# Autodesk Inventor assembly: GripperAssy
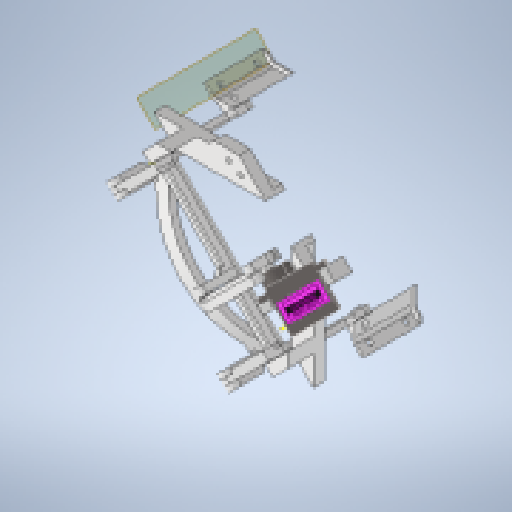
[picture p0: Inventor's stored thumbnail of the model, 512x512]
Saved by Autodesk Inventor 2025.1 (Build 291241000, 241)
## iProperties
Created: 2026-05-06
Part Number: GripperAssy
Document SubType Name: Assembly
Designer: User
Author: User
## Documents named in this file (13)
- D:\One Drive\OneDrive - Politeknik Sultan Salahuddin Abdul Aziz Shah\Documents\Inventor\RobosotPSA\GripperAssy.iam
- D:\One Drive\OneDrive - Politeknik Sultan Salahuddin Abdul Aziz Shah\Documents\Inventor\RobosotPSA\Dribbler_v2.ipt
- D:\One Drive\OneDrive - Politeknik Sultan Salahuddin Abdul Aziz Shah\Documents\Inventor\RobosotPSA\M90S_ali\M90S_ali\M90S_ali.ipt
- D:\One Drive\OneDrive - Politeknik Sultan Salahuddin Abdul Aziz Shah\Documents\Inventor\RobosotPSA\MG90S_arm01\MG90S_arm01\MG90S_arm01.ipt
- D:\One Drive\OneDrive - Politeknik Sultan Salahuddin Abdul Aziz Shah\Documents\Inventor\RobosotPSA\Gripper.ipt
- D:\One Drive\OneDrive - Politeknik Sultan Salahuddin Abdul Aziz Shah\Documents\Inventor\RobosotPSA\ServoShaft.ipt
- D:\One Drive\OneDrive - Politeknik Sultan Salahuddin Abdul Aziz Shah\Documents\Inventor\RobosotPSA\GripperHandleRight.ipt
- D:\One Drive\OneDrive - Politeknik Sultan Salahuddin Abdul Aziz Shah\Documents\Inventor\RobosotPSA\GripperHandleLeft.ipt
- D:\One Drive\OneDrive - Politeknik Sultan Salahuddin Abdul Aziz Shah\Documents\Inventor\RobosotPSA\Gripper_v1.ipt
- D:\One Drive\OneDrive - Politeknik Sultan Salahuddin Abdul Aziz Shah\Documents\Inventor\RobosotPSA\GripperShaftRight.ipt
- D:\One Drive\OneDrive - Politeknik Sultan Salahuddin Abdul Aziz Shah\Documents\Inventor\RobosotPSA\GripperShaftLeft.ipt
- D:\One Drive\OneDrive - Politeknik Sultan Salahuddin Abdul Aziz Shah\Documents\Inventor\RobosotPSA\ServoShaft_v2.ipt
- D:\One Drive\OneDrive - Politeknik Sultan Salahuddin Abdul Aziz Shah\Documents\Inventor\RobosotPSA\GripperLeft.ipt
## Components (12 placed, 12 different names)
1. Dribbler_v2:1 — Flush:2, Mate:9, Mate:10
2. M90S_ali:1 — Mate:2, Mate:3, Flush:2
3. MG90S_arm01:1 — Mate:2, Mate:3, Mate:7, Mate:8, Mate:21, Mate:22
4. ServoShaft:2 — Mate:7, Mate:8, Mate:11
5. GripperHandleRight:1 — Flush:3, Flush:4, Mate:16
6. GripperHandleLeft:1 — Flush:3
7. Gripper:1 — Mate:9, Mate:10, Mate:11, Mate:12, Mate:13, Mate:14, Mate:15, Mate:23, Mate:25
8. GripperShaftLeft:1 — Mate:12, Mate:13, Mate:18
9. GripperShaftRight:1 — Mate:14, Mate:15, Mate:17
10. Gripper_v1:1 — Flush:4, Mate:16, Mate:17, Mate:18
11. ServoShaft_v2:1 — Mate:23, Mate:24, Mate:25
12. GripperLeft:1 — Mate:21, Mate:22, Mate:24
## Relationships (22: Mate 19, Flush 3)
- Mate:2 (2 mm): M90S_ali:1 ↔ MG90S_arm01:1
- Mate:3: M90S_ali:1 ↔ MG90S_arm01:1
- Flush:2: Dribbler_v2:1 ↔ M90S_ali:1
- Mate:7: MG90S_arm01:1 ↔ ServoShaft:2
- Mate:8 (0.5 mm): MG90S_arm01:1 ↔ ServoShaft:2
- Flush:3: GripperHandleRight:1 ↔ GripperHandleLeft:1
- Mate:9 (0.5 mm): Dribbler_v2:1 ↔ Gripper:1
- Mate:10: Dribbler_v2:1 ↔ Gripper:1
- Mate:11: ServoShaft:2 ↔ Gripper:1
- Mate:12: Gripper:1 ↔ GripperShaftLeft:1
- Mate:13: Gripper:1 ↔ GripperShaftLeft:1
- Mate:14: Gripper:1 ↔ GripperShaftRight:1
- Mate:15: Gripper:1 ↔ GripperShaftRight:1
- Flush:4: GripperHandleRight:1 ↔ Gripper_v1:1
- Mate:16: GripperHandleRight:1 ↔ Gripper_v1:1
- Mate:17: GripperShaftRight:1 ↔ Gripper_v1:1
- Mate:18: GripperShaftLeft:1 ↔ Gripper_v1:1
- Mate:21: MG90S_arm01:1 ↔ GripperLeft:1
- Mate:22: MG90S_arm01:1 ↔ GripperLeft:1
- Mate:23 (0.5 mm): Gripper:1 ↔ ServoShaft_v2:1
- Mate:24: ServoShaft_v2:1 ↔ GripperLeft:1
- Mate:25: Gripper:1 ↔ ServoShaft_v2:1
